# Autodesk Inventor assembly: FINAL
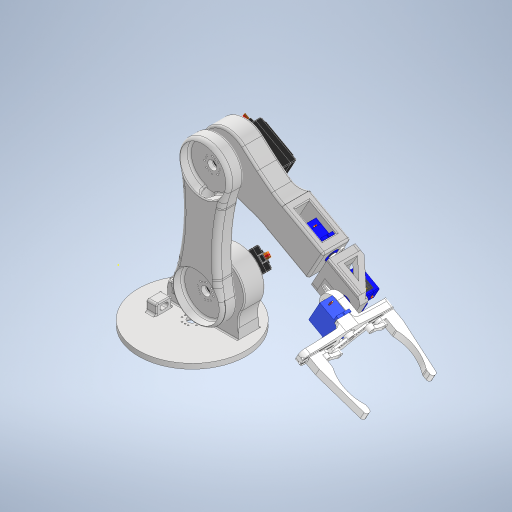
[picture p0: Inventor's stored thumbnail of the model, 512x512]
Saved by Autodesk Inventor 2024 (Build 280153000, 153)
## iProperties
Created: 2024-02-08
Part Number: FINAL
Document SubType Name: Assembly
Designer: jebes windows
Author: jebes windows
## Documents named in this file (8)
- C:\Users\jebes windows\Documents\Inventor\Robotska_roka\FINAL.iam
- C:\Users\jebes windows\Documents\Inventor\Robotska_roka\miza.ipt
- C:\Users\jebes windows\Documents\Inventor\Robotska_roka\servo-motor-mg996r-1.snapshot.1(2)\Servo Motor MG996R  With Attachments\Servo Motor MG996R  With Attachments.iam
- C:\Users\jebes windows\Documents\Inventor\Robotska_roka\roka2.ipt
- C:\Users\jebes windows\Documents\Inventor\Robotska_roka\roka1.ipt
- C:\Users\jebes windows\Documents\Inventor\Robotska_roka\sg90-micro-servo-9g-tower-pro-1.snapshot.3\SG90 - Micro Servo 9g - Tower Pro\SG90 - Micro Servo 9g - Tower Pro.iam
- C:\Users\jebes windows\Documents\Inventor\Robotska_roka\roka3.ipt
- C:\Users\jebes windows\Documents\Inventor\Robotska_roka\linear-gripper-1.snapshot.4\Linear Gripper\GRIPPER.iam
## Components (11 placed, 7 different names)
1. miza:1 — Insert:1, Angle:1
2. Servo Motor MG996R  With Attachments:1 [sub-assembly] — Insert:1, Angle:1, Insert:2
3. Servo Motor MG996R  With Attachments:2 [sub-assembly] — Insert:2, Mate:1, Mate:2, Mate:3
4. roka2:1 — Mate:7, Mate:8, Angle:2, Mate:9, Mate:10, Angle:3
5. roka1:1 — Mate:1, Mate:2, Mate:3, Mate:4, Mate:5, Mate:6
6. Servo Motor MG996R  With Attachments:3 [sub-assembly] — Mate:4, Mate:5, Mate:6, Insert:3
7. Servo Motor MG996R  With Attachments:4 [sub-assembly] — Mate:7, Mate:8, Angle:2, Insert:3
8. SG90 - Micro Servo 9g - Tower Pro:1 [sub-assembly] — Mate:9, Mate:10, Angle:3, Mate:11, Mate:12, Mate:13
9. roka3:1 — Mate:11, Mate:12, Mate:13, Mate:14, Mate:15, Angle:4, Angle:5
10. GRIPPER:1 [sub-assembly] — Mate:16, Mate:17, Angle:5
11. SG90 - Micro Servo 9g - Tower Pro:2 [sub-assembly] — Mate:14, Mate:15, Angle:4, Mate:16, Mate:17
## Relationships (25: Mate 17, Angle 5, Insert 3)
- Insert:1: miza:1 ↔ Servo Motor MG996R  With Attachments:1
- Angle:1 (90 deg): miza:1 ↔ Servo Motor MG996R  With Attachments:1
- Insert:2: Servo Motor MG996R  With Attachments:1 ↔ Servo Motor MG996R  With Attachments:2
- Mate:1: Servo Motor MG996R  With Attachments:2 ↔ roka1:1
- Mate:2: Servo Motor MG996R  With Attachments:2 ↔ roka1:1
- Mate:3: Servo Motor MG996R  With Attachments:2 ↔ roka1:1
- Mate:4: roka1:1 ↔ Servo Motor MG996R  With Attachments:3
- Mate:5: roka1:1 ↔ Servo Motor MG996R  With Attachments:3
- Mate:6: roka1:1 ↔ Servo Motor MG996R  With Attachments:3
- Mate:7: roka2:1 ↔ Servo Motor MG996R  With Attachments:4
- Mate:8: roka2:1 ↔ Servo Motor MG996R  With Attachments:4
- Angle:2 (0 deg): roka2:1 ↔ Servo Motor MG996R  With Attachments:4
- Insert:3: Servo Motor MG996R  With Attachments:3 ↔ Servo Motor MG996R  With Attachments:4
- Mate:9: roka2:1 ↔ SG90 - Micro Servo 9g - Tower Pro:1
- Mate:10: roka2:1 ↔ SG90 - Micro Servo 9g - Tower Pro:1
- Angle:3 (0 deg): roka2:1 ↔ SG90 - Micro Servo 9g - Tower Pro:1
- Mate:11: SG90 - Micro Servo 9g - Tower Pro:1 ↔ roka3:1
- Mate:12: SG90 - Micro Servo 9g - Tower Pro:1 ↔ roka3:1
- Mate:13: SG90 - Micro Servo 9g - Tower Pro:1 ↔ roka3:1
- Mate:14: roka3:1 ↔ SG90 - Micro Servo 9g - Tower Pro:2
- Mate:15: roka3:1 ↔ SG90 - Micro Servo 9g - Tower Pro:2
- Angle:4 (0 deg): roka3:1 ↔ SG90 - Micro Servo 9g - Tower Pro:2
- Mate:16: GRIPPER:1 ↔ SG90 - Micro Servo 9g - Tower Pro:2
- Mate:17: GRIPPER:1 ↔ SG90 - Micro Servo 9g - Tower Pro:2
- Angle:5 (0 deg): roka3:1 ↔ GRIPPER:1
